# Autodesk Inventor assembly: TR1 Actuator
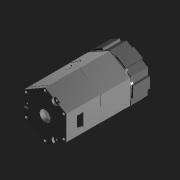
[picture p0: Inventor's stored thumbnail of the model, 180x180]
Saved by Autodesk Inventor 2017 (Build 210142000, 142)
## iProperties
Created: 2018-10-09
Part Number: TR1 Actuator
Document SubType Name: Assembly
Designer: Zach
Author: Zach
## Documents named in this file (22)
- C:\Users\Dell\Documents\GitHub\tr2\Actuator 1.4\Actuator 1.4.iam
- C:\Users\Dell\Documents\GitHub\tr2\Actuator 1.4\TA01.ipt
- C:\Users\Dell\Documents\GitHub\tr2\Actuator 1.4\EMS22XXX-D28-LSX.ipt
- C:\Users\Dell\Documents\GitHub\tr2\Actuator 1.4\12RPM Gear Motor.ipt
- C:\Users\Dell\Documents\GitHub\tr2\Actuator 1.4\Slip Ring.ipt
- C:\Users\Dell\Documents\GitHub\tr2\Actuator 1.4\TA06.ipt
- C:\Users\Dell\Documents\GitHub\tr2\Actuator 1.4\Steel Tubing.ipt
- C:\Users\Dell\Documents\GitHub\tr2\Actuator 1.4\Flange Bearing.ipt
- C:\Users\Dell\Documents\GitHub\tr2\Actuator 1.4\Shaft Collar.ipt
- C:\Users\Dell\Documents\GitHub\tr2\Actuator 1.4\Arm Actuator\Design Accelerator\Spur Gear13.ipt
- C:\Users\Dell\Documents\GitHub\tr2\Actuator 1.4\6mm Mounting Hub, thick.ipt
- C:\Users\Dell\Documents\GitHub\tr2\Actuator 1.4\TA02c.ipt
- C:\Users\Dell\Documents\GitHub\tr2\Actuator 1.4\TA02b.ipt
- C:\Users\Dell\Documents\GitHub\tr2\Actuator 1.4\Bushing.ipt
- C:\Users\Dell\Documents\GitHub\tr2\Actuator 1.4\545340 assembly.iam
- C:\Users\Dell\Documents\GitHub\tr2\Actuator 1.4\TA07.ipt
- C:\Users\Dell\Documents\GitHub\tr2\Actuator 1.4\TA08.ipt
- C:\Users\Dell\Documents\GitHub\tr2\Actuator 1.4\Rubber Square 1 in.ipt
- C:\Users\Dell\Documents\GitHub\tr2\Actuator 1.4\TA11.ipt
- C:\Users\Dell\Documents\GitHub\tr2\Actuator 1.4\Ball Bearing 0.25in.ipt
- C:\Users\Dell\Documents\GitHub\tr2\Actuator 1.4\Thrust Bearing, Gear.ipt
- C:\Users\Dell\Documents\GitHub\tr2\Actuator 1.4\Top Cover Gear.ipt
## Components (34 placed, 21 different names)
1. TA01:1 — Mate:130, Mate:161, Mate:184, Mate:197, Mate:198, Mate:199
2. TA06:1 — Mate:34, Mate:35, Mate:82, Mate:83, Mate:215, Mate:216
3. 12RPM Gear Motor:1 — Mate:86, Mate:88, Mate:102, Mate:103, Mate:115
4. EMS22XXX-D28-LSX:1 — Mate:126, Angle:1, Mate:134, Mate:218
5. Slip Ring:1 — Mate:34, Mate:35, Mate:83
6. Steel Tubing:1 — Mate:76, Mate:77, Flush:2, Mate:82, Mate:84, Mate:96, Mate:98, Mate:104, Mate:120, Mate:162, Mate:210, Mate:212
7. Flange Bearing:1 — Mate:76, Mate:179
8. Shaft Collar:1 — Mate:77, Flush:2, Mate:180
9. Flange Bearing:2 — Mate:84, Mate:180
10. Spur Gear1:1 — Mate:88, Mate:116
11. 6mm Mounting Hub, thick:1 — Mate:86, Mate:116, Flush:3, Mate:219
12. TA02c:1 — Mate:98, Mate:99, Mate:105, Mate:127, Mate:128, Mate:130, Mate:131, Angle:2, Mate:197, Mate:198, Mate:199, Mate:200, Mate:201, Mate:202, Mate:203, Mate:205, Mate:206, Mate:207, Mate:208
13. TA02b:1 — Mate:96, Mate:99, Mate:102, Mate:103, Mate:115, Mate:126, Angle:1, Mate:131, Mate:132, Mate:133, Mate:134, Mate:179, Mate:185, Mate:187, Mate:188, Mate:189, Mate:190, Mate:191, Mate:193, Mate:194, Mate:195, Mate:196, Mate:211, Mate:219
14. Bushing:1 — Mate:104, Mate:105
15. Spur Gear1:2 — Mate:119
16. 6mm Mounting Hub, thick:2 — Mate:119, Mate:218, Flush:3
17. 545340 assembly:1 [sub-assembly] — Mate:120, Mate:214
18. EMS22XXX-D28-LSX:2 — Mate:127, Mate:128, Angle:2, Mate:135
19. TA07:1 — Mate:132, Mate:133, Mate:136, Mate:183
20. TA08:1 — Mate:135, Mate:136, Mate:183
21. Rubber Square 1 in:1 — Mate:192, Mate:193, Mate:194
22. Rubber Square 1 in:2 — Mate:186, Mate:195, Mate:196
23. TA11:1 — Mate:185, Mate:186, Mate:187, Mate:188
24. TA11:2 — Mate:189, Mate:190, Mate:191, Mate:192
25. Ball Bearing 0.25in:1 — Mate:200
26. Ball Bearing 0.25in:2 — Mate:202
27. Ball Bearing 0.25in:3 — Mate:205
28. Ball Bearing 0.25in:4 — Mate:207
29. Ball Bearing 0.25in:5 — Mate:206
30. Ball Bearing 0.25in:7 — Mate:203
31. Ball Bearing 0.25in:8 — Mate:201
32. Ball Bearing 0.25in:9 — Mate:208
33. Thrust Bearing, Gear:1 — Mate:210, Mate:211, Mate:213
34. Top Cover Gear:1 — Mate:212, Mate:213, Mate:214, Mate:215, Mate:216
## Relationships (73: Mate 69, Flush 2, Angle 2)
- Mate:34: TA06:1 ↔ Slip Ring:1
- Mate:35: TA06:1 ↔ Slip Ring:1
- Mate:76: Steel Tubing:1 ↔ Flange Bearing:1
- Mate:77: Steel Tubing:1 ↔ Shaft Collar:1
- Flush:2: Steel Tubing:1 ↔ Shaft Collar:1
- Mate:82: TA06:1 ↔ Steel Tubing:1
- Mate:83: TA06:1 ↔ Slip Ring:1
- Mate:84: Steel Tubing:1 ↔ Flange Bearing:2
- Mate:86: 12RPM Gear Motor:1 ↔ 6mm Mounting Hub, thick:1
- Mate:88: 12RPM Gear Motor:1 ↔ Spur Gear1:1
- Mate:96: Steel Tubing:1 ↔ TA02b:1
- Mate:98: Steel Tubing:1 ↔ TA02c:1
- Mate:99: TA02c:1 ↔ TA02b:1
- Mate:102: 12RPM Gear Motor:1 ↔ TA02b:1
- Mate:103: 12RPM Gear Motor:1 ↔ TA02b:1
- Mate:104: Steel Tubing:1 ↔ Bushing:1
- Mate:105: TA02c:1 ↔ Bushing:1
- Mate:115: 12RPM Gear Motor:1 ↔ TA02b:1
- Mate:116: Spur Gear1:1 ↔ 6mm Mounting Hub, thick:1
- [Mate]: Spur Gear1:2 ↔ 6mm Mounting Hub, thick:2
- Mate:119: Spur Gear1:2 ↔ 6mm Mounting Hub, thick:2
- Mate:120: Steel Tubing:1 ↔ 545340 assembly:1
- Mate:126: EMS22XXX-D28-LSX:1 ↔ TA02b:1
- Angle:1 (0 deg): EMS22XXX-D28-LSX:1 ↔ TA02b:1
- Mate:127: TA02c:1 ↔ EMS22XXX-D28-LSX:2
- Mate:128: TA02c:1 ↔ EMS22XXX-D28-LSX:2
- Mate:130: TA01:1 ↔ TA02c:1
- Mate:131: TA02c:1 ↔ TA02b:1
- Angle:2 (0 deg): TA02c:1 ↔ EMS22XXX-D28-LSX:2
- Mate:132: TA02b:1 ↔ TA07:1
- Mate:133: TA02b:1 ↔ TA07:1
- Mate:134: EMS22XXX-D28-LSX:1 ↔ TA02b:1
- Mate:135: EMS22XXX-D28-LSX:2 ↔ TA08:1
- Mate:136: TA07:1 ↔ TA08:1
- Mate:161: TA01:1
- Mate:162: Steel Tubing:1
- Mate:179: Flange Bearing:1 ↔ TA02b:1
- Mate:180: Shaft Collar:1 ↔ Flange Bearing:2
- Mate:183: TA07:1 ↔ TA08:1
- Mate:184: TA01:1
- Mate:185: TA02b:1 ↔ TA11:1
- Mate:186: Rubber Square 1 in:2 ↔ TA11:1
- Mate:187: TA02b:1 ↔ TA11:1
- Mate:188: TA02b:1 ↔ TA11:1
- Mate:189: TA02b:1 ↔ TA11:2
- Mate:190: TA02b:1 ↔ TA11:2
- Mate:191: TA02b:1 ↔ TA11:2
- Mate:192: Rubber Square 1 in:1 ↔ TA11:2
- Mate:193: TA02b:1 ↔ Rubber Square 1 in:1
- Mate:194: TA02b:1 ↔ Rubber Square 1 in:1
- Mate:195: TA02b:1 ↔ Rubber Square 1 in:2
- Mate:196: TA02b:1 ↔ Rubber Square 1 in:2
- Mate:197: TA01:1 ↔ TA02c:1
- Mate:198: TA01:1 ↔ TA02c:1
- Mate:199: TA01:1 ↔ TA02c:1
- Mate:200: TA02c:1 ↔ Ball Bearing 0.25in:1
- Mate:201: TA02c:1 ↔ Ball Bearing 0.25in:8
- Mate:202: TA02c:1 ↔ Ball Bearing 0.25in:2
- Mate:203: TA02c:1 ↔ Ball Bearing 0.25in:7
- Mate:205: TA02c:1 ↔ Ball Bearing 0.25in:3
- Mate:206: TA02c:1 ↔ Ball Bearing 0.25in:5
- Mate:207: TA02c:1 ↔ Ball Bearing 0.25in:4
- Mate:208: TA02c:1 ↔ Ball Bearing 0.25in:9
- Mate:210: Steel Tubing:1 ↔ Thrust Bearing, Gear:1
- Mate:211: TA02b:1 ↔ Thrust Bearing, Gear:1
- Mate:212: Steel Tubing:1 ↔ Top Cover Gear:1
- Mate:213: Thrust Bearing, Gear:1 ↔ Top Cover Gear:1
- Mate:214: 545340 assembly:1 ↔ Top Cover Gear:1
- Mate:215: TA06:1 ↔ Top Cover Gear:1
- Mate:216: TA06:1 ↔ Top Cover Gear:1
- Mate:218: EMS22XXX-D28-LSX:1 ↔ 6mm Mounting Hub, thick:2
- Flush:3: 6mm Mounting Hub, thick:1 ↔ 6mm Mounting Hub, thick:2
- Mate:219: 6mm Mounting Hub, thick:1 ↔ TA02b:1
## Named parameters: d140_d139 = 0 mm
